# Autodesk Inventor assembly: Simple door with glass Skeleton
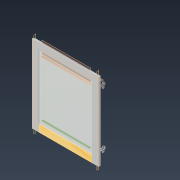
[picture p0: Inventor's stored thumbnail of the model, 180x180]
Saved by Autodesk Inventor 2022 (Build 260153000, 153)
## iProperties
RuleStatus: InUse
Created: 2017-04-13
Part Number: Simple door with glass Skeleton
Document SubType Name: Assembly
Designer: SvetlanaB
Author: SvetlanaB
## iProperties of the stored document MemberDocs/xAaaaaedaAaaaaaaaAaaaq0ztCe
RuleStatus: InUse
Created: 2017-04-13
Part Number: Simple door with glass Skeleton
Document SubType Name: Assembly
Designer: SvetlanaB
Author: SvetlanaB
## Documents named in this file (22)
- C:\W4INV 2024 Design\iBOX LIBRARY\Kitchen\Doors\One door with glass\One door with glass.iam
- C:\W4INV 2022 Design\iBOX LIBRARY\Kitchen\Doors\One door with glass\Left_panel.ipt
- C:\W4INV 2022 Design\iBOX LIBRARY\Kitchen\Doors\One door with glass\Right_panel.ipt
- C:\W4INV 2022 Design\iBOX LIBRARY\Kitchen\Doors\One door with glass\Bottom_panel.ipt
- C:\W4INV 2022 Design\iBOX LIBRARY\Kitchen\Doors\One door with glass\Top_panel.ipt
- C:\W4INV 2022 Design\iBOX LIBRARY\Kitchen\Doors\One door with glass\Glass.ipt
- C:\W4INV 2022 Design\iBOX LIBRARY\Kitchen\Doors\One door with glass\Simple door with glass Skeleton.ipt
- C:\W4INV 2022 Design\_LIBRARY\Hinges\CONCEALED HINGE\Full Overlay Hinge Wood Screw Cup Wood Screw T18.iam
- C:\W4INV 2022 Design\_LIBRARY\Fixed joints\Dowel\DOWEL V2\Dowel 8x30 PB T=18.ipt
- C:\W4INV 2021 Design\LIBRARY\Hinges\CONCEALED HINGE.iam
- C:\W4INV 2021 Design\LIBRARY\Fixed joints\Dowel\DOWEL V2.ipt
- C:\W4INV 2024 Design\iBOX LIBRARY\Kitchen\Doors\One door with glass\Left_panel.ipt
- C:\W4INV 2024 Design\iBOX LIBRARY\Kitchen\Doors\One door with glass\Right_panel.ipt
- C:\W4INV 2024 Design\iBOX LIBRARY\Kitchen\Doors\One door with glass\Bottom_panel.ipt
- C:\W4INV 2024 Design\iBOX LIBRARY\Kitchen\Doors\One door with glass\Top_panel.ipt
- C:\W4INV 2024 Design\iBOX LIBRARY\Kitchen\Doors\One door with glass\Glass.ipt
- C:\W4INV 2024 Design\iBOX LIBRARY\Kitchen\Doors\One door with glass\Simple door with glass Skeleton.ipt
- C:\W4INV 2024 Design\_LIBRARY\Hinges\CONCEALED HINGE\Full Overlay Hinge Wood Screw Cup Wood Screw T18.iam
- C:\W4INV 2024 Design\_LIBRARY\Fixed joints\Dowel\DOWEL V2\Dowel 8x30 PB T=18.ipt
- C:\W4INV 2023 Design\LIBRARY\Hinges\CONCEALED HINGE.iam
- C:\W4INV 2023 Design\LIBRARY\Fixed joints\Dowel\DOWEL V2.ipt
- C:\W4INV 2022 Design\iBOX LIBRARY\Kitchen\Doors\One door with glass\One door with glass.iam
## Components (16 placed, 8 different names)
1. @Skeleton
2. Left_panel:1 — Flush:4, Pillar Board Plane:3, Pillar Board Plane:4, Pillar Board Plane:7, Pillar Board Plane:8
3. Right_panel:1 — Flush:3, Mate:1, Mate:3, Flush:9, Pillar Board Plane:1, Pillar Board Plane:2, Pillar Board Plane:5, Pillar Board Plane:6
4. Bottom_panel:1 — Flush:2, Flush:15, Flush:16, Nestled Board Plane:5, Nestled Board Plane:6, Nestled Board Plane:7, Nestled Board Plane:8
5. Top_panel:1 — Flush:1, Flush:11, Flush:14, Nestled Board Plane:1, Nestled Board Plane:2, Nestled Board Plane:3, Nestled Board Plane:4
6. Glass:1
7. Full Overlay Hinge Wood Screw Cup Wood Screw T18:1 [sub-assembly] — Mate:1, Right top hinge, Mate:2, Left top hinge
8. Full Overlay Hinge Wood Screw Cup Wood Screw T18:2 [sub-assembly] — Mate:3, Right bottom hinge, Mate:4, Left bottom hinge
9. Dowel 8x30 PB T=18:1 — Nestled Board Plane:1, Axis Plane:1, Second Axis Plane:1, Pillar Board Plane:1
10. Dowel 8x30 PB T=18:2 — Nestled Board Plane:2, Axis Plane:2, Second Axis Plane:2, Pillar Board Plane:2
11. Dowel 8x30 PB T=18:3 — Nestled Board Plane:3, Axis Plane:3, Second Axis Plane:3, Pillar Board Plane:4
12. Dowel 8x30 PB T=18:4 — Nestled Board Plane:4, Axis Plane:4, Second Axis Plane:4, Pillar Board Plane:3
13. Dowel 8x30 PB T=18:7 — Nestled Board Plane:5, Axis Plane:5, Second Axis Plane:5, Pillar Board Plane:5
14. Dowel 8x30 PB T=18:8 — Nestled Board Plane:6, Axis Plane:6, Second Axis Plane:6, Pillar Board Plane:6
15. Dowel 8x30 PB T=18:9 — Nestled Board Plane:7, Axis Plane:7, Second Axis Plane:7, Pillar Board Plane:7
16. Dowel 8x30 PB T=18:10 — Nestled Board Plane:8, Axis Plane:8, Second Axis Plane:8, Pillar Board Plane:8
## Relationships (49: Mate 36, Flush 13)
- Flush:1 (-100 mm): Top_panel:1
- Flush:2 (-100 mm): Bottom_panel:1
- Flush:3 (-16.5 mm): Right_panel:1
- Flush:4 (-16.5 mm): Left_panel:1
- Mate:1: Right_panel:1 ↔ Full Overlay Hinge Wood Screw Cup Wood Screw T18:1
- Right top hinge [Flush]: Full Overlay Hinge Wood Screw Cup Wood Screw T18:1
- Mate:2: Full Overlay Hinge Wood Screw Cup Wood Screw T18:1
- Mate:3: Right_panel:1 ↔ Full Overlay Hinge Wood Screw Cup Wood Screw T18:2
- Right bottom hinge [Flush]: Full Overlay Hinge Wood Screw Cup Wood Screw T18:2
- Mate:4: Full Overlay Hinge Wood Screw Cup Wood Screw T18:2
- Flush:9 (-20 mm): Right_panel:1
- Flush:11 (-9 mm): Top_panel:1
- Flush:14 (-20 mm): Top_panel:1
- Flush:15 (-20 mm): Bottom_panel:1
- Flush:16 (-20 mm): Bottom_panel:1
- Left top hinge [Flush]: Full Overlay Hinge Wood Screw Cup Wood Screw T18:1
- Left bottom hinge [Flush]: Full Overlay Hinge Wood Screw Cup Wood Screw T18:2
- Nestled Board Plane:1 [Mate]: Top_panel:1 ↔ Dowel 8x30 PB T=18:1
- Axis Plane:1 [Mate]: Dowel 8x30 PB T=18:1
- Second Axis Plane:1 [Mate]: Dowel 8x30 PB T=18:1
- Nestled Board Plane:2 [Mate]: Top_panel:1 ↔ Dowel 8x30 PB T=18:2
- Axis Plane:2 [Mate]: Dowel 8x30 PB T=18:2
- Second Axis Plane:2 [Mate]: Dowel 8x30 PB T=18:2
- Pillar Board Plane:1 [Mate] (-9 mm): Right_panel:1 ↔ Dowel 8x30 PB T=18:1
- Pillar Board Plane:2 [Mate] (-9 mm): Right_panel:1 ↔ Dowel 8x30 PB T=18:2
- Nestled Board Plane:3 [Mate]: Top_panel:1 ↔ Dowel 8x30 PB T=18:3
- Axis Plane:3 [Mate]: Dowel 8x30 PB T=18:3
- Second Axis Plane:3 [Mate]: Dowel 8x30 PB T=18:3
- Nestled Board Plane:4 [Mate]: Top_panel:1 ↔ Dowel 8x30 PB T=18:4
- Axis Plane:4 [Mate]: Dowel 8x30 PB T=18:4
- Second Axis Plane:4 [Mate]: Dowel 8x30 PB T=18:4
- Pillar Board Plane:3 [Mate] (-9 mm): Left_panel:1 ↔ Dowel 8x30 PB T=18:4
- Pillar Board Plane:4 [Mate] (-9 mm): Left_panel:1 ↔ Dowel 8x30 PB T=18:3
- Nestled Board Plane:5 [Mate]: Bottom_panel:1 ↔ Dowel 8x30 PB T=18:7
- Axis Plane:5 [Mate]: Dowel 8x30 PB T=18:7
- Second Axis Plane:5 [Mate]: Dowel 8x30 PB T=18:7
- Nestled Board Plane:6 [Mate]: Bottom_panel:1 ↔ Dowel 8x30 PB T=18:8
- Axis Plane:6 [Mate]: Dowel 8x30 PB T=18:8
- Second Axis Plane:6 [Mate]: Dowel 8x30 PB T=18:8
- Pillar Board Plane:5 [Mate] (-9 mm): Right_panel:1 ↔ Dowel 8x30 PB T=18:7
- Pillar Board Plane:6 [Mate] (-9 mm): Right_panel:1 ↔ Dowel 8x30 PB T=18:8
- Nestled Board Plane:7 [Mate]: Bottom_panel:1 ↔ Dowel 8x30 PB T=18:9
- Axis Plane:7 [Mate]: Dowel 8x30 PB T=18:9
- Second Axis Plane:7 [Mate]: Dowel 8x30 PB T=18:9
- Nestled Board Plane:8 [Mate]: Bottom_panel:1 ↔ Dowel 8x30 PB T=18:10
- Axis Plane:8 [Mate]: Dowel 8x30 PB T=18:10
- Second Axis Plane:8 [Mate]: Dowel 8x30 PB T=18:10
- Pillar Board Plane:7 [Mate] (-9 mm): Left_panel:1 ↔ Dowel 8x30 PB T=18:9
- Pillar Board Plane:8 [Mate] (-9 mm): Left_panel:1 ↔ Dowel 8x30 PB T=18:10
## Named parameters: Panel_thickness = 18 mm, Left_offset = 1.5 mm, Right_offset = 1.5 mm, Top_offset = 1.5 mm, Bottom_offset = 1.5 mm, Front_offset = 2 mm, Cupboard_Panel_Thickness = 18 mm, Hinge_top_offset = 100 mm, Hinge_bottom_offset = 100 mm, Width = 600 mm, Depth = 400 mm, Height = 700 mm, Type = 1, Carcass_thickness = 60 mm
